# Autodesk Inventor assembly: BasePruebasSensores
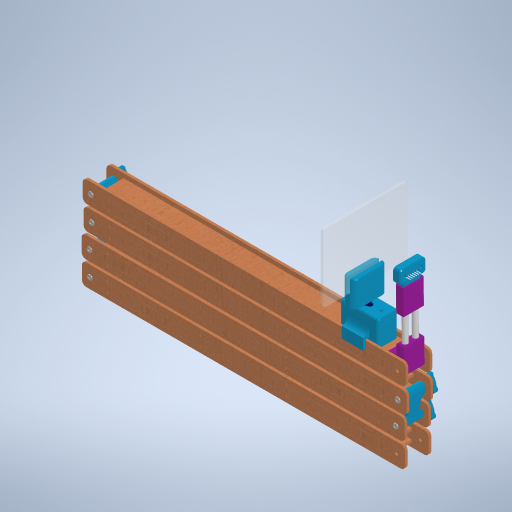
[picture p0: Inventor's stored thumbnail of the model, 512x512]
Saved by Autodesk Inventor 2024 (Build 280153000, 153)
## iProperties
Created: 2023-11-01
Part Number: BasePruebasSensores
Document SubType Name: Assembly
Designer: fredy
Author: fredy
## Documents named in this file (17)
- D:\UVG_1Ciclo_2023\Tesis\Tesis_WS_FredyGodoy19260\BasePruebasSensores\BasePruebasSensores.iam
- D:\UVG_1Ciclo_2023\Tesis\Tesis_WS_FredyGodoy19260\BasePruebasSensores\Pared.ipt
- D:\UVG_1Ciclo_2023\Tesis\Tesis_WS_FredyGodoy19260\BasePruebasSensores\ConectorPared.ipt
- D:\UVG_1Ciclo_2023\Tesis\Tesis_WS_FredyGodoy19260\BasePruebasSensores\ConectorBrazos.ipt
- D:\UVG_1Ciclo_2023\Tesis\Tesis_WS_FredyGodoy19260\BasePruebasSensores\Sensores\VL53L0X TOF Sensor Distancia\VL53L0X TOF Sensor Distancia.ipt
- D:\UVG_1Ciclo_2023\Tesis\Tesis_WS_FredyGodoy19260\BasePruebasSensores\Base_VL53L0X.ipt
- D:\UVG_1Ciclo_2023\Tesis\Tesis_WS_FredyGodoy19260\BasePruebasSensores\Servo\MicroServo-SG90\MicroServo-SG90.ipt
- D:\UVG_1Ciclo_2023\Tesis\Tesis_WS_FredyGodoy19260\BasePruebasSensores\BaseRotativa.ipt
- D:\UVG_1Ciclo_2023\Tesis\Tesis_WS_FredyGodoy19260\BasePruebasSensores\Servo\Microservo horn\Microservo horn.ipt
- D:\UVG_1Ciclo_2023\Tesis\Tesis_WS_FredyGodoy19260\BasePruebasSensores\Base_MaterialRotativo.ipt
- D:\UVG_1Ciclo_2023\Tesis\Tesis_WS_FredyGodoy19260\BasePruebasSensores\PlacaObjetivo.ipt
- D:\UVG_1Ciclo_2023\Tesis\Tesis_WS_FredyGodoy19260\BasePruebasSensores\BaseAux_Sensor_V2_PInferior.ipt
- D:\UVG_1Ciclo_2023\Tesis\Tesis_WS_FredyGodoy19260\BasePruebasSensores\BaseAux_Sensor_V2_PSuperior.ipt
- D:\UVG_1Ciclo_2023\Tesis\Tesis_WS_FredyGodoy19260\BasePruebasSensores\PerfilTubular_BaseSensor.ipt
- D:\UVG_1Ciclo_2023\Tesis\Tesis_WS_FredyGodoy19260\BasePruebasSensores\CubreTuerca.ipt
- C:\Users\fredy\OneDrive\Documents\Inventor\Content Center Files\R2024\en-US\AS 1427(05)\AS 1427 - M3 x 40(5) II.ipt
- C:\Users\fredy\OneDrive\Documents\Inventor\Content Center Files\R2024\en-US\AS 1112 (2)\AS 1112 - M3  Type 5.ipt
## Components (48 placed, 16 different names)
1. Pared:1 — Mate:1, Mate:2, Mate:3, Mate:4
2. ConectorPared:1 — Mate:1, Mate:2, Mate:5, Mate:6, Mate:39
3. ConectorPared:2 — Mate:3, Mate:4
4. Pared:2 — Mate:5, Mate:6, Insert:1, Insert:17, Mate:20, Insert:22
5. Pared:3
6. ConectorPared:3
7. ConectorPared:4
8. Pared:4 — Insert:2, Insert:14, Insert:23, Insert:26
9. ConectorBrazos:1 — Insert:1, Insert:2
10. VL53L0X TOF Sensor Distancia:1 — Insert:3, Insert:4
11. Base_VL53L0X:1 — Insert:3, Insert:4, Mate:37, Mate:38
12. MicroServo-SG90:1 — Insert:8, Insert:11, Insert:12
13. BaseRotativa:1 — Mate:20, Insert:11, Insert:12, Mate:39
14. Microservo horn:1 — Insert:8, Insert:9, Insert:10
15. Base_MaterialRotativo:1 — Insert:9, Insert:10, Mate:22, Mate:23, Mate:24
16. PlacaObjetivo:1 — Mate:22, Mate:23, Mate:24
17. Pared:5
18. ConectorPared:5
19. ConectorPared:6
20. Pared:6 — Insert:16, Insert:24, Insert:27
21. ConectorBrazos:2 — Insert:14
22. Pared:7
23. ConectorPared:7
24. ConectorPared:8
25. Pared:8 — Insert:25
26. ConectorBrazos:3 — Insert:16
27. BaseAux_Sensor_V2_PInferior:1 — Insert:17, Insert:20, Insert:21
28. BaseAux_Sensor_V2_PSuperior:1 — Mate:37, Mate:38, Insert:18, Insert:19
29. PerfilTubular_BaseSensor:1 — Insert:18, Insert:20
30. PerfilTubular_BaseSensor:2 — Insert:19, Insert:21
31. AS 1427 H - Metric M3 x 40:4 — Insert:26, Insert:40
32. AS 1427 H - Metric M3 x 40:1 — Insert:24, Insert:38
33. AS 1427 H - Metric M3 x 40:6 — Insert:22, Insert:42
34. AS 1427 H - Metric M3 x 40:5 — Insert:27, Insert:41
35. AS 1427 H - Metric M3 x 40:3 — Insert:25, Insert:39
36. AS 1427 H - Metric M3 x 40:2 — Insert:23, Insert:37
37. CubreTuerca:8 — Insert:28, Insert:42
38. AS 1112 (2) - Metric M3  Type 5:1 — Insert:28
39. CubreTuerca:9 — Insert:37
40. AS 1112 (2) - Metric M3  Type 5:2
41. CubreTuerca:10 — Insert:40
42. AS 1112 (2) - Metric M3  Type 5:3
43. CubreTuerca:11 — Insert:39
44. AS 1112 (2) - Metric M3  Type 5:4
45. CubreTuerca:12 — Insert:41
46. AS 1112 (2) - Metric M3  Type 5:5
47. CubreTuerca:13 — Insert:38
48. AS 1112 (2) - Metric M3  Type 5:6
## Relationships (67: Insert 36, Mate 31)
- Mate:1: Pared:1 ↔ ConectorPared:1
- Mate:2: Pared:1 ↔ ConectorPared:1
- Mate:3: Pared:1 ↔ ConectorPared:2
- Mate:4: Pared:1 ↔ ConectorPared:2
- Mate:5: ConectorPared:1 ↔ Pared:2
- Mate:6: ConectorPared:1 ↔ Pared:2
- [Mate]: Pared:3 ↔ ConectorPared:3
- [Mate]: Pared:3 ↔ ConectorPared:3
- [Mate]: Pared:3 ↔ ConectorPared:4
- [Mate]: Pared:3 ↔ ConectorPared:4
- [Mate]: ConectorPared:3 ↔ Pared:4
- [Mate]: ConectorPared:3 ↔ Pared:4
- Insert:1: Pared:2 ↔ ConectorBrazos:1
- Insert:2: Pared:4 ↔ ConectorBrazos:1
- Insert:3: VL53L0X TOF Sensor Distancia:1 ↔ Base_VL53L0X:1
- Insert:4: VL53L0X TOF Sensor Distancia:1 ↔ Base_VL53L0X:1
- Mate:20 (0.5 mm): Pared:2 ↔ BaseRotativa:1
- Insert:8: MicroServo-SG90:1 ↔ Microservo horn:1
- Insert:9: Microservo horn:1 ↔ Base_MaterialRotativo:1
- Insert:10: Microservo horn:1 ↔ Base_MaterialRotativo:1
- Insert:11: MicroServo-SG90:1 ↔ BaseRotativa:1
- Insert:12: MicroServo-SG90:1 ↔ BaseRotativa:1
- Mate:22: Base_MaterialRotativo:1 ↔ PlacaObjetivo:1
- Mate:23: Base_MaterialRotativo:1 ↔ PlacaObjetivo:1
- Mate:24: Base_MaterialRotativo:1 ↔ PlacaObjetivo:1
- [Mate]: Pared:5 ↔ ConectorPared:5
- [Mate]: Pared:5 ↔ ConectorPared:5
- [Mate]: Pared:5 ↔ ConectorPared:6
- [Mate]: Pared:5 ↔ ConectorPared:6
- [Mate]: ConectorPared:5 ↔ Pared:6
- [Mate]: ConectorPared:5 ↔ Pared:6
- [Insert]: Pared:6 ↔ ConectorBrazos:2
- Insert:14: Pared:4 ↔ ConectorBrazos:2
- [Mate]: Pared:7 ↔ ConectorPared:7
- [Mate]: Pared:7 ↔ ConectorPared:7
- [Mate]: Pared:7 ↔ ConectorPared:8
- [Mate]: Pared:7 ↔ ConectorPared:8
- [Mate]: ConectorPared:7 ↔ Pared:8
- [Mate]: ConectorPared:7 ↔ Pared:8
- [Insert]: Pared:8 ↔ ConectorBrazos:3
- Insert:16: Pared:6 ↔ ConectorBrazos:3
- Insert:17: Pared:2 ↔ BaseAux_Sensor_V2_PInferior:1
- Mate:37: Base_VL53L0X:1 ↔ BaseAux_Sensor_V2_PSuperior:1
- Mate:38: Base_VL53L0X:1 ↔ BaseAux_Sensor_V2_PSuperior:1
- Insert:18: BaseAux_Sensor_V2_PSuperior:1 ↔ PerfilTubular_BaseSensor:1
- Insert:19: BaseAux_Sensor_V2_PSuperior:1 ↔ PerfilTubular_BaseSensor:2
- Insert:20: BaseAux_Sensor_V2_PInferior:1 ↔ PerfilTubular_BaseSensor:1
- Insert:21: BaseAux_Sensor_V2_PInferior:1 ↔ PerfilTubular_BaseSensor:2
- Mate:39: ConectorPared:1 ↔ BaseRotativa:1
- Insert:22: Pared:2 ↔ AS 1427 H - Metric M3 x 40:6
- Insert:23: Pared:4 ↔ AS 1427 H - Metric M3 x 40:2
- Insert:24: Pared:6 ↔ AS 1427 H - Metric M3 x 40:1
- Insert:25: Pared:8 ↔ AS 1427 H - Metric M3 x 40:3
- Insert:26: Pared:4 ↔ AS 1427 H - Metric M3 x 40:4
- Insert:27: Pared:6 ↔ AS 1427 H - Metric M3 x 40:5
- Insert:28: CubreTuerca:8 ↔ AS 1112 (2) - Metric M3  Type 5:1
- [Insert]: CubreTuerca:9 ↔ AS 1112 (2) - Metric M3  Type 5:2
- [Insert]: CubreTuerca:10 ↔ AS 1112 (2) - Metric M3  Type 5:3
- [Insert]: CubreTuerca:11 ↔ AS 1112 (2) - Metric M3  Type 5:4
- [Insert]: CubreTuerca:12 ↔ AS 1112 (2) - Metric M3  Type 5:5
- [Insert]: CubreTuerca:13 ↔ AS 1112 (2) - Metric M3  Type 5:6
- Insert:37: AS 1427 H - Metric M3 x 40:2 ↔ CubreTuerca:9
- Insert:38: AS 1427 H - Metric M3 x 40:1 ↔ CubreTuerca:13
- Insert:39: AS 1427 H - Metric M3 x 40:3 ↔ CubreTuerca:11
- Insert:40: AS 1427 H - Metric M3 x 40:4 ↔ CubreTuerca:10
- Insert:41: AS 1427 H - Metric M3 x 40:5 ↔ CubreTuerca:12
- Insert:42: AS 1427 H - Metric M3 x 40:6 ↔ CubreTuerca:8
## Named parameters: d8_d3 = 0 mm, d9_d4 = 0 mm, d10_d5 = 0 mm, d11_d6 = 0 mm, d12_d7 = 0 mm, d13_d1 = 0 mm, d65_d8_d3 = 0 mm, d66_d9_d4 = 0 mm, d67_d10_d5 = 0 mm, d68_d11_d6 = 0 mm, d69_d12_d7 = 0 mm, d70_d13_d1 = 0 mm, d71_d15 = 0 mm, d73_d8_d3 = 0 mm, d74_d9_d4 = 0 mm, d75_d10_d5 = 0 mm, d76_d11_d6 = 0 mm, d77_d12_d7 = 0 mm, d78_d13_d1 = 0 mm, d79_d15 = 0 mm, d127_d125 = 0 mm, d129_d125 = 0 mm, d130_d125 = 0 mm, d131_d125 = 0 mm, d132_d125 = 0 mm
